# Autodesk Inventor assembly: oar_buttons2
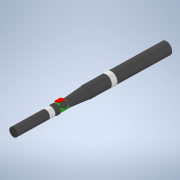
[picture p0: Inventor's stored thumbnail of the model, 180x180]
Saved by Autodesk Inventor 2020 (Build 240168000, 168)
## iProperties
Created: 2019-11-18
Part Number: oar_buttons2
Document SubType Name: Assembly
Designer: suchanek
Author: suchanek
## Documents named in this file (6)
- D:\suchanek\programming\rowing_steering\model_final\oar_buttons2.iam
- D:\suchanek\programming\rowing_steering\model_final\oar.ipt
- D:\suchanek\programming\rowing_steering\model_final\buttons2_flexible_buttons.ipt
- D:\suchanek\programming\rowing_steering\model_final\buttons_battery.ipt
- D:\suchanek\programming\rowing_steering\model_final\buttons_BLE_nano.ipt
- D:\suchanek\programming\rowing_steering\model_final\buttons2_PCBs.ipt
## Components (5 placed, 5 different names)
1. oar:1 — Flush:1, Flush:2, Flush:3, Tangent:1, Tangent:2, Mate:1
2. buttons2_flexible_buttons:1 — Flush:1, Flush:2, Flush:3
3. buttons2_PCBs:1 — Tangent:1, Tangent:2, Mate:1, Rigid:1, Rigid:2
4. buttons_battery:1 — Rigid:2
5. buttons_BLE_nano:1 — Rigid:1
## Relationships (8: Flush 3, Tangent 2, WeldJoint 2, Mate 1)
- Flush:1: oar:1 ↔ buttons2_flexible_buttons:1
- Flush:2 (10 mm): oar:1 ↔ buttons2_flexible_buttons:1
- Flush:3 (-75 mm): oar:1 ↔ buttons2_flexible_buttons:1
- Tangent:1: oar:1 ↔ buttons2_PCBs:1
- Tangent:2: oar:1 ↔ buttons2_PCBs:1
- Mate:1: oar:1 ↔ buttons2_PCBs:1
- Rigid:1 [WeldJoint]: buttons2_PCBs:1 ↔ buttons_BLE_nano:1
- Rigid:2 [WeldJoint]: buttons2_PCBs:1 ↔ buttons_battery:1
